# Autodesk Inventor assembly: Expermental Setup
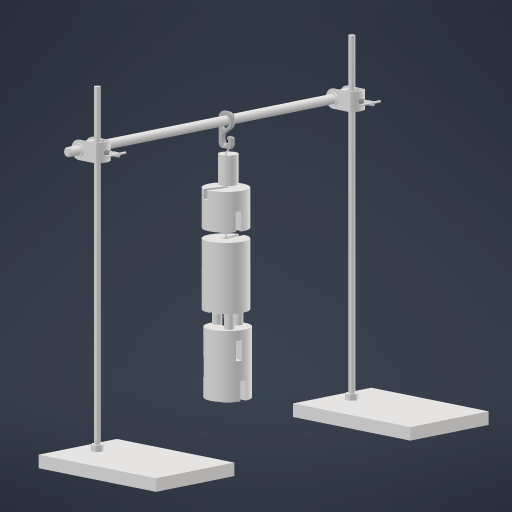
[picture p0: Inventor's stored thumbnail of the model, 512x512]
Saved by Autodesk Inventor 2023.1 (Build 271208000, 208)
## iProperties
Created: 2022-12-06
Part Number: Expermental Setup
Document SubType Name: Assembly
Designer: aubrey-work
Author: aubrey-work
## Documents named in this file (6)
- C:\GitHubRepos\PHYS-12-Website\content\portfolio\CAD Practice\Entries\3-Physics201L Test Hook Apparatus\Expermental Setup.iam
- C:\GitHubRepos\PHYS-12-Website\content\portfolio\CAD Practice\Entries\3-Physics201L Test Hook Apparatus\Ring Stand.iam
- C:\GitHubRepos\PHYS-12-Website\content\portfolio\CAD Practice\Entries\3-Physics201L Test Hook Apparatus\Metal Rod.ipt
- C:\GitHubRepos\PHYS-12-Website\content\portfolio\FRC Floor Layout\Aubreys\Graduated Shelves\Hook.ipt
- C:\GitHubRepos\PHYS-12-Website\content\portfolio\CAD Practice\Entries\3-Physics201L Test Hook Apparatus\Masses.iam
- C:\GitHubRepos\PHYS-12-Website\content\portfolio\CAD Practice\Entries\3-Physics201L Test Hook Apparatus\Test Hook for Inventor v9.ipt
## Components (6 placed, 5 different names)
1. Ring Stand:1 [sub-assembly] — Mate:2, Mate:3, Flush:1, Mate:4, Flush:2, Flush:3, Angle:3
2. Ring Stand:2 [sub-assembly] — Mate:5, Mate:6, Flush:3, Angle:1, Mate:8
3. Metal Rod:1 — Mate:4, Flush:2, Mate:5, Mate:6, Mate:7, Mate:8, Mate:10, Mate:11
4. Hook:1 — Mate:7, Angle:1, Mate:10
5. Masses:1 [sub-assembly] — Mate:13, Angle:2, Flush:13, Flush:5
6. Test Hook for Inventor v9:1 — Mate:11, Mate:13, Angle:2, Flush:13, Flush:5, Angle:3
## Relationships (18: Mate 10, Flush 5, Angle 3)
- Mate:2: Ring Stand:1
- Mate:3: Ring Stand:1
- Flush:1: Ring Stand:1
- Mate:4: Ring Stand:1 ↔ Metal Rod:1
- Flush:2 (-31.75 mm): Ring Stand:1 ↔ Metal Rod:1
- Mate:5: Ring Stand:2 ↔ Metal Rod:1
- Mate:6 (31.75 mm): Ring Stand:2 ↔ Metal Rod:1
- Flush:3: Ring Stand:1 ↔ Ring Stand:2
- Mate:7 (12.7 mm): Metal Rod:1 ↔ Hook:1
- Angle:1 (0 deg): Ring Stand:2 ↔ Hook:1
- Mate:8: Ring Stand:2 ↔ Metal Rod:1
- Mate:10: Metal Rod:1 ↔ Hook:1
- Mate:11: Metal Rod:1 ↔ Test Hook for Inventor v9:1
- Mate:13 (-2.5 mm): Masses:1 ↔ Test Hook for Inventor v9:1
- Angle:2 (0 deg): Masses:1 ↔ Test Hook for Inventor v9:1
- Flush:13 (18 mm): Masses:1 ↔ Test Hook for Inventor v9:1
- Flush:5 (7.5 mm): Masses:1 ↔ Test Hook for Inventor v9:1
- Angle:3 (0 deg): Ring Stand:1 ↔ Test Hook for Inventor v9:1
